# Autodesk Inventor assembly: top
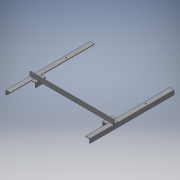
[picture p0: Inventor's stored thumbnail of the model, 180x180]
Saved by Autodesk Inventor 2017 (Build 210142000, 142)
## iProperties
Created: 2018-10-22
Part Number: top
Document SubType Name: Assembly
Designer: ddeboer
Author: ddeboer
## Documents named in this file (4)
- C:\Users\ddeboer\Desktop\snap_holder\top.iam
- C:\Users\ddeboer\Desktop\snap_holder\angle_L102.ipt
- C:\Users\ddeboer\Desktop\snap_holder\angle_S.ipt
- C:\Users\ddeboer\Desktop\snap_holder\angle_L101.ipt
## Components (5 placed, 4 different names)
1. angle_L102:front — Insert:1, Angle:1, Insert:2, Flush:1, Insert:3, Flush:2, Insert:4, Angle:2
2. angle_S:1 — Insert:1, Angle:1
3. angle_L101:right — Insert:2, Flush:1
4. angle_L101:2 — Insert:3, Flush:2
5. angle_S:2 — Insert:4, Angle:2
## Relationships (8: Insert 4, Angle 2, Flush 2)
- Insert:1: angle_L102:front ↔ angle_S:1
- Angle:1 (0 deg): angle_L102:front ↔ angle_S:1
- Insert:2: angle_L102:front ↔ angle_L101:right
- Flush:1: angle_L102:front ↔ angle_L101:right
- Insert:3: angle_L102:front ↔ angle_L101:2
- Flush:2: angle_L102:front ↔ angle_L101:2
- Insert:4: angle_L102:front ↔ angle_S:2
- Angle:2 (180 deg): angle_L102:front ↔ angle_S:2
